# Autodesk Inventor assembly: SklopReduktora
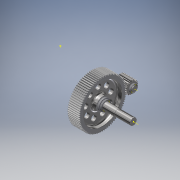
[picture p0: Inventor's stored thumbnail of the model, 180x180]
Saved by Autodesk Inventor 2018 (Build 220112000, 112)
## iProperties
Created: 2018-11-17
Part Number: SklopReduktora
Document SubType Name: Assembly
Designer: Kristijan
Mass: 76453.9 g
Surface Area: 10005.2 cm^2
Volume: 9794.09 cm^3
Density: 7.80613 g/cm^3
Author: Kristijan
## Documents named in this file (8)
- C:\Users\krist\Dropbox (Personal)\PolitehnikaPula\5 semestar\Konstrukcije\TimskiProjektniZadatak\OutputDrawings\SklopReduktora.iam
- C:\Users\krist\Dropbox (Personal)\PolitehnikaPula\5 semestar\Konstrukcije\TimskiProjektniZadatak\datasheetsModels\6008.iam
- C:\Users\krist\Dropbox (Personal)\PolitehnikaPula\5 semestar\Konstrukcije\TimskiProjektniZadatak\OutputDrawings\GonjenoVratilo.ipt
- C:\Users\krist\Dropbox (Personal)\PolitehnikaPula\5 semestar\Konstrukcije\TimskiProjektniZadatak\datasheetsModels\32913.iam
- C:\Users\krist\Dropbox (Personal)\PolitehnikaPula\5 semestar\Konstrukcije\TimskiProjektniZadatak\datasheetsModels\DIN 6885 - A 22 x 14 x 90.ipt
- C:\Users\krist\Dropbox (Personal)\PolitehnikaPula\5 semestar\Konstrukcije\TimskiProjektniZadatak\OutputDrawings\PogonskoVratiloSaZupcanikom.ipt
- C:\Users\krist\Dropbox (Personal)\PolitehnikaPula\5 semestar\Konstrukcije\TimskiProjektniZadatak\OutputDrawings\DistantniPrsten.ipt
- C:\Users\krist\Dropbox (Personal)\PolitehnikaPula\5 semestar\Konstrukcije\TimskiProjektniZadatak\OutputDrawings\GonjeniZupcanik_olaksani.ipt
## Components (9 placed, 7 different names)
1. 6008:1 [sub-assembly] — Mate:17, Mate:18
2. 6008:2 [sub-assembly] — Mate:15, Mate:16
3. GonjenoVratilo — Mate:7, Mate:8, Mate:9, Rigid:1, Flush:16, Mate:19, Mate:22
4. 32913:1 [sub-assembly] — Mate:7, Mate:21
5. 32913:2 [sub-assembly] — Mate:8, Mate:9
6. GonjeniZupcanik
7. DIN 6885-1 A A 22 x 14 x 90:1 — Rigid:1
8. Pogonsko vratilo sa zupcanikom — Mate:15, Mate:16, Mate:17, Mate:18, Flush:17, Mate:22
9. DistantniPrsten:1 — Mate:19, Mate:21
## Relationships (19: Mate 13, Flush 4, WeldJoint 1, RelateRotation 1)
- Mate:7: GonjenoVratilo ↔ 32913:1
- Mate:8: GonjenoVratilo ↔ 32913:2
- Mate:9: GonjenoVratilo ↔ 32913:2
- [Mate]: GonjenoVratilo ↔ GonjeniZupcanik
- Rigid:1 [WeldJoint]: GonjenoVratilo ↔ DIN 6885-1 A A 22 x 14 x 90:1
- [Flush]: GonjenoVratilo ↔ GonjeniZupcanik
- [Mate]: GonjenoVratilo ↔ GonjeniZupcanik
- Mate:15: 6008:2 ↔ Pogonsko vratilo sa zupcanikom
- Mate:16: 6008:2 ↔ Pogonsko vratilo sa zupcanikom
- Mate:17: 6008:1 ↔ Pogonsko vratilo sa zupcanikom
- Mate:18: 6008:1 ↔ Pogonsko vratilo sa zupcanikom
- Flush:16: GonjenoVratilo
- Flush:17: Pogonsko vratilo sa zupcanikom
- Mate:19: GonjenoVratilo ↔ DistantniPrsten:1
- [Mate]: GonjeniZupcanik ↔ DistantniPrsten:1
- [Flush] (-2.5 mm): GonjeniZupcanik ↔ Pogonsko vratilo sa zupcanikom
- Mate:21: 32913:1 ↔ DistantniPrsten:1
- [RelateRotation] (1 ul): GonjeniZupcanik ↔ Pogonsko vratilo sa zupcanikom
- Mate:22 (262.5 mm): GonjenoVratilo ↔ Pogonsko vratilo sa zupcanikom
